# Autodesk Inventor assembly: LAYOUT
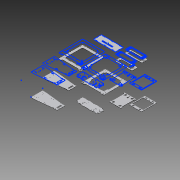
[picture p0: Inventor's stored thumbnail of the model, 180x180]
Saved by Autodesk Inventor 2013 (Build 170138000, 138)
## iProperties
Created: 2014-06-23
Part Number: LAYOUT
Document SubType Name: Assembly
Designer: employee
Author: employee
## Documents named in this file (12)
- C:\Users\employee\Desktop\CoreXZ 2\LAYOUT.iam
- C:\Users\employee\Desktop\CoreXZ 2\BACK PLATE.ipt
- C:\Users\employee\Desktop\CoreXZ 2\BED PLATE BOTTOM.ipt
- C:\Users\employee\Desktop\CoreXZ 2\BED PLATE TOP.ipt
- C:\Users\employee\Desktop\CoreXZ 2\BOTTOM PLATE.ipt
- C:\Users\employee\Desktop\CoreXZ 2\FRONT PLATE.ipt
- C:\Users\employee\Desktop\CoreXZ 2\GANTRY BACK.ipt
- C:\Users\employee\Desktop\CoreXZ 2\GANTRY FRONT.ipt
- C:\Users\employee\Desktop\CoreXZ 2\RETAINER.ipt
- C:\Users\employee\Desktop\CoreXZ 2\TOP PLATE.ipt
- C:\Users\employee\Desktop\CoreXZ 2\SIDE PLATE.ipt
- C:\Users\employee\Desktop\CoreXZ 2\layout.ipt
## Components (15 placed, 11 different names)
1. BACK PLATE:1
2. BED PLATE BOTTOM:1
3. BED PLATE TOP:1
4. BOTTOM PLATE:1
5. FRONT PLATE:1
6. GANTRY BACK:1
7. GANTRY FRONT:1
8. RETAINER:1
9. RETAINER:2
10. RETAINER:3
11. RETAINER:4
12. TOP PLATE:1 — Flush:1
13. SIDE PLATE:1
14. SIDE PLATE:2
15. layout:1 — Flush:1
## Relationships (1: Flush 1)
- Flush:1: TOP PLATE:1 ↔ layout:1
